# Autodesk Inventor assembly: Kit Frame 26x30
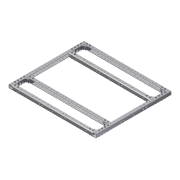
[picture p0: Inventor's stored thumbnail of the model, 180x180]
Saved by Autodesk Inventor 2013 (Build 170138000, 138)
## iProperties
Created: 2013-01-06
Part Number: Kit Frame 26x30
Document SubType Name: Assembly
Designer: Nemo
Author: Nemo
## Documents named in this file (4)
- \\lmss\STUDENTS\Robotics\CAD Files\COTS Parts\Kit Frame - AndyMark\Kit Frame 26x30.iam
- \\lmss\STUDENTS\Robotics\CAD Files\COTS Parts\Kit Frame - AndyMark\Components\24x34 Side Rail sub.iam
- \\lmss\STUDENTS\Robotics\CAD Files\COTS Parts\Kit Frame - AndyMark\Components\C Channel - FrontBack 26x30.ipt
- \\lmss\STUDENTS\Robotics\CAD Files\COTS Parts\Kit Frame - AndyMark\Components\26x30 Side Rail Sub mirror.iam
## Components (6 placed, 3 different names)
1. C Channel - Cut-01:3 — Flush:5, Mate:15
2. C Channel - Cut-01:4 — Mate:3, Mate:13, Insert:1, Mate:16, Insert:2, Mate:17, Insert:3, Mate:18
3. 24x34 Side Rail sub:1 [sub-assembly] — Mate:13, Mate:15
4. 26x30 Side Rail Sub mirror:1 [sub-assembly] — Insert:1, Mate:16
5. 24x34 Side Rail sub:2 [sub-assembly] — Insert:2, Mate:17
6. 26x30 Side Rail Sub mirror:2 [sub-assembly] — Insert:3, Mate:18
## Relationships (14: Mate 8, Flush 3, Insert 3)
- [Mate] (36.83 mm): 24x34 Side Rail sub:1
- [Mate]: 24x34 Side Rail sub:1
- [Flush]: C Channel - Cut-01:3 ↔ 24x34 Side Rail sub:1
- [Flush]: C Channel - Cut-01:4 ↔ 24x34 Side Rail sub:1
- Flush:5: C Channel - Cut-01:3
- Mate:3: C Channel - Cut-01:4
- Mate:13: C Channel - Cut-01:4 ↔ 24x34 Side Rail sub:1
- Mate:15: C Channel - Cut-01:3 ↔ 24x34 Side Rail sub:1
- Insert:1: C Channel - Cut-01:4 ↔ 26x30 Side Rail Sub mirror:1
- Mate:16: C Channel - Cut-01:4 ↔ 26x30 Side Rail Sub mirror:1
- Insert:2: C Channel - Cut-01:4 ↔ 24x34 Side Rail sub:2
- Mate:17: C Channel - Cut-01:4 ↔ 24x34 Side Rail sub:2
- Insert:3: C Channel - Cut-01:4 ↔ 26x30 Side Rail Sub mirror:2
- Mate:18: C Channel - Cut-01:4 ↔ 26x30 Side Rail Sub mirror:2
